# Autodesk Inventor assembly: ASM_Screw_Coupler
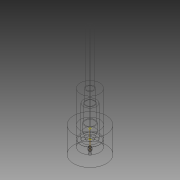
[picture p0: Inventor's stored thumbnail of the model, 180x180]
Saved by Autodesk Inventor 2011 SP2 (Build 150309200, 309)
## iProperties
Created: 2012-02-15
Part Number: ASM_Screw_Coupler
Document SubType Name: Assembly
Designer: sungwook
Author: sungwook
## Documents named in this file (6)
- C:\Users\sungwook\Documents\Inventor\Micron20\Assembly\ASM_Screw_Coupler.iam
- C:\Users\sungwook\Documents\Inventor\Micron20\Parts\Jigs\Screw_Asm_Jig_Lower.ipt
- C:\Users\sungwook\Documents\Inventor\Micron20\Parts\Jigs\Screw_Asm_Jig_Upper.ipt
- C:\Users\sungwook\Documents\Inventor\Micron20\Parts\Jigs\Collect_Jaw.ipt
- C:\Users\sungwook\Documents\Inventor\Micron20\Parts\Motor Units\MU_Motor_Coupling_3.ipt
- C:\Users\sungwook\Documents\Inventor\Micron20\Parts\Motor Units\MU_Motor_Thread.ipt
## Components (5 placed, 5 different names)
1. Screw_Asm_Jig_Lower:1 — Mate:1, Mate:2, Mate:7, Mate:8
2. Screw_Asm_Jig_Upper:1 — Mate:5, Mate:6, Mate:7, Mate:8, Flush:1
3. Collect_Jaw:1 — Mate:3, Mate:4, Mate:5, Mate:6, Flush:1
4. MU_Motor_Coupling_3:1 — Mate:1, Mate:2, Mate:9
5. MU_Motor_Thread:1 — Mate:3, Mate:4, Mate:9
## Relationships (10: Mate 9, Flush 1)
- Mate:1: Screw_Asm_Jig_Lower:1 ↔ MU_Motor_Coupling_3:1
- Mate:2: Screw_Asm_Jig_Lower:1 ↔ MU_Motor_Coupling_3:1
- Mate:3: Collect_Jaw:1 ↔ MU_Motor_Thread:1
- Mate:4: Collect_Jaw:1 ↔ MU_Motor_Thread:1
- Mate:5: Screw_Asm_Jig_Upper:1 ↔ Collect_Jaw:1
- Mate:6: Screw_Asm_Jig_Upper:1 ↔ Collect_Jaw:1
- Mate:7: Screw_Asm_Jig_Lower:1 ↔ Screw_Asm_Jig_Upper:1
- Mate:8: Screw_Asm_Jig_Lower:1 ↔ Screw_Asm_Jig_Upper:1
- Flush:1: Screw_Asm_Jig_Upper:1 ↔ Collect_Jaw:1
- Mate:9: MU_Motor_Coupling_3:1 ↔ MU_Motor_Thread:1
